# Autodesk Inventor assembly: Baugruppe1
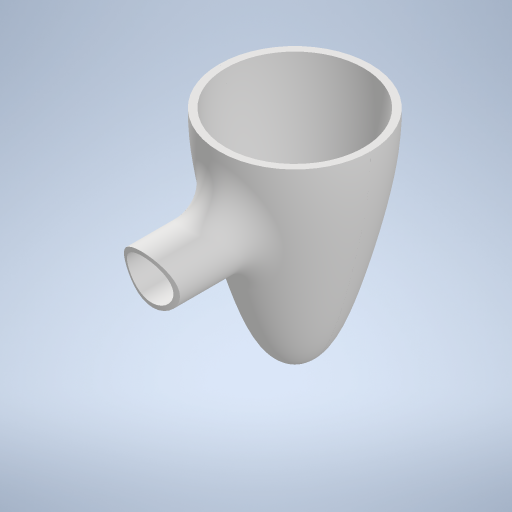
[picture p0: Inventor's stored thumbnail of the model, 512x512]
Saved by Autodesk Inventor 2023 (Build 270158000, 158)
## iProperties
Created: 2023-03-30
Part Number: Baugruppe1
Document SubType Name: Assembly
Designer: Lukas
Author: Lukas
## Documents named in this file (3)
- C:\Users\Lukas\OneDrive\Dokumente\Inventor\Baugruppe1.iam
- C:\Users\Lukas\OneDrive\Dokumente\Inventor\DeckelGehaeuse.ipt
- C:\Users\Lukas\OneDrive\Dokumente\Inventor\TurmGehaeuse.ipt
## Components (2 placed, 2 different names)
1. DeckelGehaeuse:1 — Symmetrie:1
2. TurmGehaeuse:1 — Symmetrie:1
## Relationships (1: Symmetry 1)
- Symmetrie:1: DeckelGehaeuse:1 ↔ TurmGehaeuse:1
